# Autodesk Inventor assembly: Latest Assembly
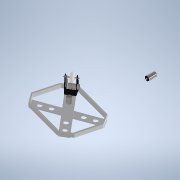
[picture p0: Inventor's stored thumbnail of the model, 180x180]
Saved by Autodesk Inventor 2020 (Build 240168000, 168)
## iProperties
Created: 2022-07-18
Part Number: Latest Assembly
Document SubType Name: Assembly
Designer: karimi2
Author: karimi2
## Documents named in this file (4)
- C:\Users\karimi2\Documents\PROJECT\src\Latest Assembly.iam
- C:\Users\karimi2\Documents\PROJECT\src\Wheel Assembly.iam
- C:\Users\karimi2\Documents\PROJECT\src\New Chassis.ipt
- C:\Users\karimi2\Documents\PROJECT\src\GearedDCmotor.ipt
## Components (4 placed, 3 different names)
1. Wheel Assembly:1 [sub-assembly] — Mate:1, Rotational:1
2. New Chassis:1 — Mate:1, Rotational:1, Mate:2, Rigid:1
3. GearedDCmotor:1 — Mate:2, Rigid:1
4. GearedDCmotor:2
## Relationships (4: Mate 2, RevoluteJoint 1, WeldJoint 1)
- Mate:1: Wheel Assembly:1 ↔ New Chassis:1
- Rotational:1 [RevoluteJoint] (-5 mm): Wheel Assembly:1 ↔ New Chassis:1
- Mate:2: New Chassis:1 ↔ GearedDCmotor:1
- Rigid:1 [WeldJoint]: New Chassis:1 ↔ GearedDCmotor:1
